# Autodesk Inventor assembly: Electrical Board 1
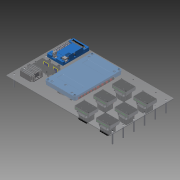
[picture p0: Inventor's stored thumbnail of the model, 180x180]
Saved by Autodesk Inventor 2013 (Build 170138000, 138)
## iProperties
Created: 2013-01-27
Part Number: Electrical Board 1
Document SubType Name: Assembly
Designer: Moses
Mass: 2458.26 g
Surface Area: 9144.76 cm^2
Volume: 1395.98 cm^3
Density: 1.76095 g/cm^3
Author: Moses
## Documents named in this file (8)
- C:\Users\Arpan\Documents\GitHub\frc2013CAD\Electrical\Electrical Board 1.iam
- C:\Users\Arpan\Documents\GitHub\frc2013CAD\Electrical\Mounting Board 1.ipt
- C:\Users\Arpan\Documents\GitHub\frc2013CAD\Electrical\CS_PowerBoard_A003206.ipt
- C:\Users\Arpan\Documents\GitHub\frc2013CAD\Electrical\CS_Converter_CLL25-24S05.ipt
- C:\Users\Arpan\Documents\GitHub\frc2013CAD\Electrical\93330A493\93330A493.ipt
- C:\Users\Arpan\Documents\GitHub\frc2013CAD\Electrical\CS_Relay_SPIKE-RELAY-H.ipt
- C:\Users\Arpan\Documents\GitHub\frc2013CAD\Electrical\Talon with Fan.iam
- C:\Users\Arpan\Documents\GitHub\frc2013CAD\Electrical\CS_SideCar_A003333.ipt
## Components (23 placed, 7 different names)
1. Mounting Board 1:1 — Mate:1, Mate:2, Mate:3, Mate:4, Mate:5, Mate:6, Mate:7, Mate:8, Mate:9, Mate:10, Mate:11, Mate:12, Mate:13, Mate:14, Mate:15, Mate:16, Mate:17, Mate:18, Mate:19, Mate:20, Mate:21, Mate:22, Mate:23, Mate:24, Mate:25, Mate:26, Insert:2, Insert:4, Insert:5, Insert:6, Insert:7, Insert:8, Mate:27, Mate:28, Mate:29, Mate:30, Mate:31, Mate:32, Mate:33, Mate:34, Mate:35, Insert:9, Insert:10, Insert:11, Insert:12, Insert:13
2. Talon with Fan:1 [sub-assembly] — Mate:1, Mate:6, Mate:7
3. Talon with Fan:2 [sub-assembly] — Mate:2, Mate:8, Mate:9
4. Talon with Fan:3 [sub-assembly] — Mate:3, Mate:10, Mate:11
5. Talon with Fan:4 [sub-assembly] — Mate:4, Mate:12, Mate:13
6. Talon with Fan:5 [sub-assembly] — Mate:14, Mate:15, Mate:16
7. Talon with Fan:6 [sub-assembly] — Mate:5, Mate:17, Mate:18
8. CS_PowerBoard_A003206:1 — Mate:19, Mate:20, Mate:21, Mate:22, Mate:23
9. CS_Converter_CLL25-24S05:1 — Mate:24, Mate:25, Mate:26
10. 93330A493:2 — Insert:2
11. 93330A493:4 — Insert:4
12. 93330A493:5 — Insert:5
13. 93330A493:6 — Insert:6
14. 93330A493:7 — Insert:7
15. 93330A493:8 — Insert:8
16. CS_Relay_SPIKE-RELAY-H:1 — Mate:28, Mate:29, Mate:30
17. CS_Relay_SPIKE-RELAY-H:2 — Mate:27, Mate:31, Mate:32
18. CS_SideCar_A003333:1 — Mate:33, Mate:34, Mate:35
19. 93330A493:9 — Insert:10
20. 93330A493:10 — Insert:9
21. 93330A493:11 — Insert:11
22. 93330A493:12 — Insert:12
23. 93330A493:13 — Insert:13
## Relationships (46: Mate 35, Insert 11)
- Mate:1: Mounting Board 1:1 ↔ Talon with Fan:1
- Mate:2: Mounting Board 1:1 ↔ Talon with Fan:2
- Mate:3: Mounting Board 1:1 ↔ Talon with Fan:3
- Mate:4: Mounting Board 1:1 ↔ Talon with Fan:4
- Mate:5: Mounting Board 1:1 ↔ Talon with Fan:6
- Mate:6: Mounting Board 1:1 ↔ Talon with Fan:1
- Mate:7: Mounting Board 1:1 ↔ Talon with Fan:1
- Mate:8: Mounting Board 1:1 ↔ Talon with Fan:2
- Mate:9: Mounting Board 1:1 ↔ Talon with Fan:2
- Mate:10: Mounting Board 1:1 ↔ Talon with Fan:3
- Mate:11: Mounting Board 1:1 ↔ Talon with Fan:3
- Mate:12: Mounting Board 1:1 ↔ Talon with Fan:4
- Mate:13: Mounting Board 1:1 ↔ Talon with Fan:4
- Mate:14: Mounting Board 1:1 ↔ Talon with Fan:5
- Mate:15: Mounting Board 1:1 ↔ Talon with Fan:5
- Mate:16: Mounting Board 1:1 ↔ Talon with Fan:5
- Mate:17: Mounting Board 1:1 ↔ Talon with Fan:6
- Mate:18: Mounting Board 1:1 ↔ Talon with Fan:6
- Mate:19: Mounting Board 1:1 ↔ CS_PowerBoard_A003206:1
- Mate:20: Mounting Board 1:1 ↔ CS_PowerBoard_A003206:1
- Mate:21: Mounting Board 1:1 ↔ CS_PowerBoard_A003206:1
- Mate:22: Mounting Board 1:1 ↔ CS_PowerBoard_A003206:1
- Mate:23: Mounting Board 1:1 ↔ CS_PowerBoard_A003206:1
- Mate:24: Mounting Board 1:1 ↔ CS_Converter_CLL25-24S05:1
- Mate:25: Mounting Board 1:1 ↔ CS_Converter_CLL25-24S05:1
- Mate:26: Mounting Board 1:1 ↔ CS_Converter_CLL25-24S05:1
- Insert:2: Mounting Board 1:1 ↔ 93330A493:2
- Insert:4: Mounting Board 1:1 ↔ 93330A493:4
- Insert:5: Mounting Board 1:1 ↔ 93330A493:5
- Insert:6: Mounting Board 1:1 ↔ 93330A493:6
- Insert:7: Mounting Board 1:1 ↔ 93330A493:7
- Insert:8: Mounting Board 1:1 ↔ 93330A493:8
- Mate:27: Mounting Board 1:1 ↔ CS_Relay_SPIKE-RELAY-H:2
- Mate:28: Mounting Board 1:1 ↔ CS_Relay_SPIKE-RELAY-H:1
- Mate:29: Mounting Board 1:1 ↔ CS_Relay_SPIKE-RELAY-H:1
- Mate:30: Mounting Board 1:1 ↔ CS_Relay_SPIKE-RELAY-H:1
- Mate:31: Mounting Board 1:1 ↔ CS_Relay_SPIKE-RELAY-H:2
- Mate:32: Mounting Board 1:1 ↔ CS_Relay_SPIKE-RELAY-H:2
- Mate:33: Mounting Board 1:1 ↔ CS_SideCar_A003333:1
- Mate:34: Mounting Board 1:1 ↔ CS_SideCar_A003333:1
- Mate:35: Mounting Board 1:1 ↔ CS_SideCar_A003333:1
- Insert:9: Mounting Board 1:1 ↔ 93330A493:10
- Insert:10: Mounting Board 1:1 ↔ 93330A493:9
- Insert:11: Mounting Board 1:1 ↔ 93330A493:11
- Insert:12: Mounting Board 1:1 ↔ 93330A493:12
- Insert:13: Mounting Board 1:1 ↔ 93330A493:13
